# Autodesk Inventor assembly: 3mm-nozzle-assembly
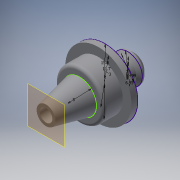
[picture p0: Inventor's stored thumbnail of the model, 180x180]
Saved by Autodesk Inventor 2017 (Build 210142000, 142)
## iProperties
Created: 2026-03-25
Part Number: 3mm-nozzle-assembly
Document SubType Name: Assembly
Designer: a
Author: a
## Documents named in this file (3)
- C:\Users\a\Documents\the-claw-pnp\3mm-nozzle-assembly.iam
- C:\Users\a\Documents\the-claw-pnp\juki-head-assembly.iam
- C:\Users\a\Documents\the-claw-pnp\nozzle-3mm-tip.ipt
## Components (2 placed, 2 different names)
1. juki-head-assembly:1 [sub-assembly] — Mate:1, Mate:2
2. nozzle-3mm-tip:1 — Mate:1, Mate:2
## Relationships (2: Mate 2)
- Mate:1: juki-head-assembly:1 ↔ nozzle-3mm-tip:1
- Mate:2: juki-head-assembly:1 ↔ nozzle-3mm-tip:1
